# Autodesk Inventor assembly: Ensemble_Boite_chassis
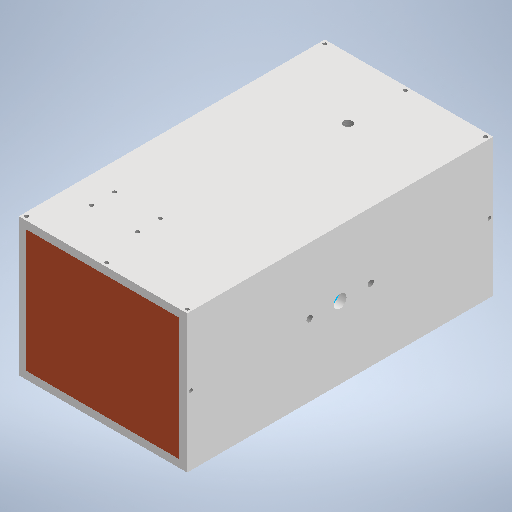
[picture p0: Inventor's stored thumbnail of the model, 512x512]
Saved by Autodesk Inventor 2026.2 (Build 302298010, 298A)
## iProperties
Created: 2026-03-16
Part Number: Ensemble_Boite_chassis
Document SubType Name: Assembly
Designer: genon
Author: genon
## Documents named in this file (8)
- C:\Users\genon\Documents\Henallux Passerelle\Projet de conception\Cassini T-X\Inventor\Ensemble_Boite_chassis.iam
- C:\Users\genon\Documents\Henallux Passerelle\Projet de conception\Cassini T-X\Inventor\chassis_bas.ipt
- C:\Users\genon\Documents\Henallux Passerelle\Projet de conception\Cassini T-X\Inventor\chassis_côté.ipt
- C:\Users\genon\Documents\Henallux Passerelle\Projet de conception\Cassini T-X\Inventor\chassis_face_arriere.ipt
- C:\Users\genon\Documents\Henallux Passerelle\Projet de conception\Cassini T-X\Inventor\chassis_haut.ipt
- C:\Users\genon\Documents\Henallux Passerelle\Projet de conception\Cassini T-X\Inventor\Composants\Arduino Mega 2560\Arduino Mega 2560\Arduino Mega 2560.ipt
- C:\Users\genon\Documents\Henallux Passerelle\Projet de conception\Cassini T-X\Inventor\Composants\Batterie.ipt
- C:\Users\genon\Documents\Henallux Passerelle\Projet de conception\Cassini T-X\Inventor\chassis arriere.ipt
## Components (8 placed, 7 different names)
1. chassis_bas:1 — Placage:1, Placage:2, Placage:3, Placage:4, Placage:5, Placage:11, Placage:12
2. chassis_côté:1 — Placage:1, Placage:2, Placage:6
3. chassis_côté:2 — Placage:3, Placage:4, Placage:9, Placage:13
4. chassis_face_arriere:2 — Placage:5, Placage:6, Placage:10
5. chassis_haut:1 — Placage:9, Placage:10, Placage:14
6. Arduino Mega 2560:1 — Placage:12
7. Batterie:1 — Placage:11
8. chassis arriere:1 — Placage:13, Placage:14
## Relationships (12: Mate 12)
- Placage:1 [Mate]: chassis_bas:1 ↔ chassis_côté:1
- Placage:2 [Mate]: chassis_bas:1 ↔ chassis_côté:1
- Placage:3 [Mate]: chassis_bas:1 ↔ chassis_côté:2
- Placage:4 [Mate]: chassis_bas:1 ↔ chassis_côté:2
- Placage:5 [Mate]: chassis_bas:1 ↔ chassis_face_arriere:2
- Placage:6 [Mate]: chassis_côté:1 ↔ chassis_face_arriere:2
- Placage:9 [Mate]: chassis_côté:2 ↔ chassis_haut:1
- Placage:10 [Mate]: chassis_face_arriere:2 ↔ chassis_haut:1
- Placage:11 [Mate]: chassis_bas:1 ↔ Batterie:1
- Placage:12 [Mate]: chassis_bas:1 ↔ Arduino Mega 2560:1
- Placage:13 [Mate]: chassis_côté:2 ↔ chassis arriere:1
- Placage:14 [Mate]: chassis_haut:1 ↔ chassis arriere:1
